# Autodesk Inventor assembly: 3DCP-NOZZLE
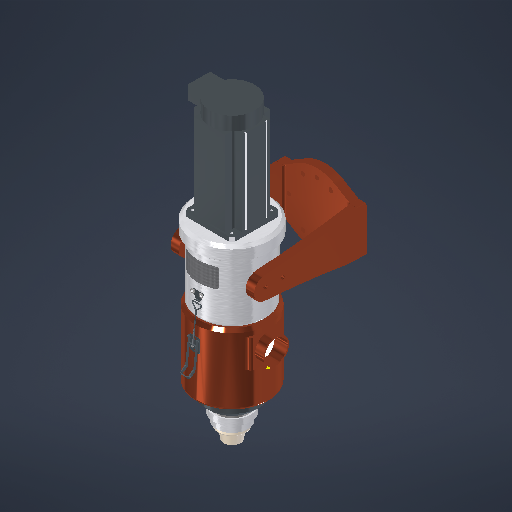
[picture p0: Inventor's stored thumbnail of the model, 512x512]
Saved by Autodesk Inventor 2025.3 (Build 293356030, 356C)
## iProperties
Created: 2025-08-29
Part Number: 3DCP-NOZZLE
Document SubType Name: Assembly
Designer: lstk1ng
Description: EXTRUSOR DE CONCRETO
Mass: 2977.25 g
Surface Area: 5747.16 cm^2
Volume: 2874.48 cm^3
Density: 1.03575 g/cm^3
Author: lstk1ng
Revision Number: 1.0
## Documents named in this file (13)
- C:\Users\lstk1ng\Documents\UPC\UPC-10\PROYECTO MECATRONICO 1\DISEÑO MECANICO\3DCP-NOZZLE.iam
- C:\Users\lstk1ng\Documents\UPC\UPC-10\PROYECTO MECATRONICO 1\DISEÑO MECANICO\UPPER-NOZZLE.ipt
- C:\Users\lstk1ng\Documents\UPC\UPC-10\PROYECTO MECATRONICO 1\DISEÑO MECANICO\LOWER-NOZZLEv2.ipt
- C:\Users\lstk1ng\Documents\UPC\UPC-10\PROYECTO MECATRONICO 1\DISEÑO MECANICO\MOUNTING-COUPLE.ipt
- C:\Users\lstk1ng\Documents\UPC\UPC-10\PROYECTO MECATRONICO 1\DISEÑO MECANICO\HOSE-NOZZLE-MOUNTING.ipt
- C:\Users\lstk1ng\Documents\UPC\UPC-10\PROYECTO MECATRONICO 1\DISEÑO MECANICO\220LB LOCK\HEAD-220LB.ipt
- C:\Users\lstk1ng\Documents\Inventor\Content Center Files\R2025\en-US\IFI 513(8)\IFI 513 - M4x0.7 x 8(4) II.ipt
- C:\Users\lstk1ng\Documents\UPC\UPC-10\PROYECTO MECATRONICO 1\DISEÑO MECANICO\220LB LOCK\220LB-ASSY.iam
- C:\Users\lstk1ng\Documents\UPC\UPC-10\PROYECTO MECATRONICO 1\DISEÑO MECANICO\EXTRUSSOR-COUPLING.ipt
- C:\Users\lstk1ng\Documents\UPC\UPC-10\PROYECTO MECATRONICO 1\DISEÑO MECANICO\NOZZLE-EXTRUSOR.ipt
- C:\Users\lstk1ng\Documents\UPC\UPC-10\PROYECTO MECATRONICO 1\DISEÑO MECANICO\COMPONENTS\SERVOMOTOR-1KW.ipt
- C:\Users\lstk1ng\Documents\UPC\UPC-10\PROYECTO MECATRONICO 1\DISEÑO MECANICO\AUGER-SCREW.ipt
- C:\Users\lstk1ng\Documents\UPC\UPC-10\PROYECTO MECATRONICO 1\DISEÑO MECANICO\COMPONENTS\JAW-COUPLING.ipt
## Components (17 placed, 12 different names)
1. LOWER-NOZZLEv2:1 — Insert:4, Insert:7, Insert:8
2. UPPER-NOZZLE:2 — Insert:4, Cylindrical:1, Cylindrical:2, Cylindrical:3, Mate:4, Mate:5, Mate:6, Tangent:1, Mate:7, Mate:8
3. HOSE-NOZZLE-MOUNTING:1
4. MOUNTING-COUPLE:1 — Tangent:1, Mate:7, Mate:8
5. HEAD-220LB:1 — Insert:2, Insert:3
6. 220LB-ASSY:1 [sub-assembly]
7. HEAD-220LB:2 — Insert:5, Insert:6
8. 220LB-ASSY:2 [sub-assembly]
9. EXTRUSSOR-COUPLING:1 — Insert:7
10. NOZZLE-EXTRUSOR:1 — Insert:8
11. SERVOMOTOR-1KW:1 — Mate:4, Mate:5, Mate:6, Insert:9
12. AUGER-SCREW:1 — Insert:10, Angle:1
13. JAW-COUPLING:1 — Insert:9, Insert:10
14. Square Recessed Oval Countersunk Head Machine Screw - Type III - Metric (2) M4x0.7 x 8:5 — Insert:5, Cylindrical:3
15. Square Recessed Oval Countersunk Head Machine Screw - Type III - Metric (2) M4x0.7 x 8:4 — Insert:6
16. Square Recessed Oval Countersunk Head Machine Screw - Type III - Metric (2) M4x0.7 x 8:3 — Insert:3, Cylindrical:2
17. Square Recessed Oval Countersunk Head Machine Screw - Type III - Metric (2) M4x0.7 x 8:2 — Insert:2, Cylindrical:1
## Relationships (19: Insert 9, Mate 5, CylindricalJoint 3, Tangent 1, Angle 1)
- Insert:2: HEAD-220LB:1 ↔ Square Recessed Oval Countersunk Head Machine Screw - Type III - Metric (2) M4x0.7 x 8:2
- Insert:3: HEAD-220LB:1 ↔ Square Recessed Oval Countersunk Head Machine Screw - Type III - Metric (2) M4x0.7 x 8:3
- Insert:4: LOWER-NOZZLEv2:1 ↔ UPPER-NOZZLE:2
- Cylindrical:1: UPPER-NOZZLE:2 ↔ Square Recessed Oval Countersunk Head Machine Screw - Type III - Metric (2) M4x0.7 x 8:2
- Cylindrical:2: UPPER-NOZZLE:2 ↔ Square Recessed Oval Countersunk Head Machine Screw - Type III - Metric (2) M4x0.7 x 8:3
- Insert:5: HEAD-220LB:2 ↔ Square Recessed Oval Countersunk Head Machine Screw - Type III - Metric (2) M4x0.7 x 8:5
- Insert:6: HEAD-220LB:2 ↔ Square Recessed Oval Countersunk Head Machine Screw - Type III - Metric (2) M4x0.7 x 8:4
- Cylindrical:3: UPPER-NOZZLE:2 ↔ Square Recessed Oval Countersunk Head Machine Screw - Type III - Metric (2) M4x0.7 x 8:5
- Insert:7: LOWER-NOZZLEv2:1 ↔ EXTRUSSOR-COUPLING:1
- Insert:8: LOWER-NOZZLEv2:1 ↔ NOZZLE-EXTRUSOR:1
- Mate:4: UPPER-NOZZLE:2 ↔ SERVOMOTOR-1KW:1
- Mate:5: UPPER-NOZZLE:2 ↔ SERVOMOTOR-1KW:1
- Mate:6: UPPER-NOZZLE:2 ↔ SERVOMOTOR-1KW:1
- Tangent:1: UPPER-NOZZLE:2 ↔ MOUNTING-COUPLE:1
- Mate:7: UPPER-NOZZLE:2 ↔ MOUNTING-COUPLE:1
- Mate:8: UPPER-NOZZLE:2 ↔ MOUNTING-COUPLE:1
- Insert:9: SERVOMOTOR-1KW:1 ↔ JAW-COUPLING:1
- Insert:10: AUGER-SCREW:1 ↔ JAW-COUPLING:1
- Angle:1 (-1000 deg): AUGER-SCREW:1
